# Autodesk Inventor assembly: sistema embebido
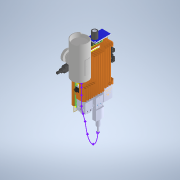
[picture p0: Inventor's stored thumbnail of the model, 180x180]
Saved by Autodesk Inventor 2021 (Build 250183000, 183)
## iProperties
Created: 2022-12-03
Part Number: sistema embebido
Document SubType Name: Assembly
Designer: user
Author: user
## Documents named in this file (9)
- D:\ESPOL\Tesis\3d proto\Total\sistema embebido.iam
- D:\ESPOL\Tesis\3d proto\Total\Assembly Raspberry Pi 4 B.iam
- D:\ESPOL\Tesis\3d proto\Total\Heat sink.ipt
- D:\ESPOL\Tesis\3d proto\Total\Heatsink Base.ipt
- D:\ESPOL\Tesis\3d proto\Total\MLX90640.ipt
- D:\ESPOL\Tesis\3d proto\Total\camara hd.ipt
- D:\ESPOL\Tesis\3d proto\Total\cable usb.ipt
- D:\ESPOL\Tesis\3d proto\Total\USB C.ipt
- D:\ESPOL\Tesis\3d proto\Total\jumper.ipt
## Components (21 placed, 8 different names)
1. Assembly Raspberry Pi 4 B:1 [sub-assembly] — Coincidencia:1, Coincidencia:2, Nivelación:1, Nivelación:2, Nivelación:3, Nivelación:4, Coincidencia:3, Coincidencia:4, Coincidencia:5, Coincidencia:10, Coincidencia:11, Coincidencia:17, Coincidencia:18, Coincidencia:19, Coincidencia:20, Coincidencia:21, Coincidencia:22, Coincidencia:23, Coincidencia:24, Coincidencia:25, Coincidencia:26, Coincidencia:27, Coincidencia:28, Coincidencia:29, Coincidencia:30, Coincidencia:31, Coincidencia:32, Coincidencia:33, Coincidencia:34, Coincidencia:35, Coincidencia:36
2. Heat sink:1 — Coincidencia:2, Nivelación:1, Nivelación:4
3. Heatsink Base:1 — Coincidencia:1, Nivelación:2, Nivelación:3, Coincidencia:37
4. MLX90640:1 — Coincidencia:3, Coincidencia:12, Coincidencia:13, Coincidencia:14, Coincidencia:15
5. camara hd:1 — Coincidencia:6, Coincidencia:37
6. cable usb:1 — Coincidencia:4, Coincidencia:5, Coincidencia:7
7. USB C:1 — Coincidencia:10, Coincidencia:11
8. jumper:1 — Coincidencia:15
9. jumper:2 — Coincidencia:14
10. jumper:3 — Coincidencia:13
11. jumper:4 — Coincidencia:23, Coincidencia:24
12. jumper:5 — Coincidencia:25, Coincidencia:26
13. jumper:6 — Coincidencia:27, Coincidencia:28
14. jumper:7 — Coincidencia:19, Coincidencia:20
15. jumper:8 — Coincidencia:12
16. jumper:9 — Coincidencia:21, Coincidencia:22
17. jumper:10 — Coincidencia:17, Coincidencia:18
18. jumper:11 — Coincidencia:31, Coincidencia:32
19. jumper:12 — Coincidencia:33, Coincidencia:34
20. jumper:13 — Coincidencia:35, Coincidencia:36
21. jumper:14 — Coincidencia:29, Coincidencia:30
## Relationships (40: Mate 36, Flush 4)
- Coincidencia:1 [Mate]: Assembly Raspberry Pi 4 B:1 ↔ Heatsink Base:1
- Coincidencia:2 [Mate]: Assembly Raspberry Pi 4 B:1 ↔ Heat sink:1
- Nivelación:1 [Flush]: Assembly Raspberry Pi 4 B:1 ↔ Heat sink:1
- Nivelación:2 [Flush]: Assembly Raspberry Pi 4 B:1 ↔ Heatsink Base:1
- Nivelación:3 [Flush]: Assembly Raspberry Pi 4 B:1 ↔ Heatsink Base:1
- Nivelación:4 [Flush]: Assembly Raspberry Pi 4 B:1 ↔ Heat sink:1
- Coincidencia:3 [Mate] (20 mm): Assembly Raspberry Pi 4 B:1 ↔ MLX90640:1
- Coincidencia:4 [Mate]: Assembly Raspberry Pi 4 B:1 ↔ cable usb:1
- Coincidencia:5 [Mate]: Assembly Raspberry Pi 4 B:1 ↔ cable usb:1
- Coincidencia:6 [Mate]: camara hd:1
- Coincidencia:7 [Mate]: cable usb:1
- Coincidencia:8 [Mate]
- Coincidencia:9 [Mate]
- Coincidencia:10 [Mate]: Assembly Raspberry Pi 4 B:1 ↔ USB C:1
- Coincidencia:11 [Mate]: Assembly Raspberry Pi 4 B:1 ↔ USB C:1
- Coincidencia:12 [Mate]: MLX90640:1 ↔ jumper:8
- Coincidencia:13 [Mate]: MLX90640:1 ↔ jumper:3
- Coincidencia:14 [Mate]: MLX90640:1 ↔ jumper:2
- Coincidencia:15 [Mate]: MLX90640:1 ↔ jumper:1
- Coincidencia:17 [Mate]: Assembly Raspberry Pi 4 B:1 ↔ jumper:10
- Coincidencia:18 [Mate]: Assembly Raspberry Pi 4 B:1 ↔ jumper:10
- Coincidencia:19 [Mate]: Assembly Raspberry Pi 4 B:1 ↔ jumper:7
- Coincidencia:20 [Mate]: Assembly Raspberry Pi 4 B:1 ↔ jumper:7
- Coincidencia:21 [Mate]: Assembly Raspberry Pi 4 B:1 ↔ jumper:9
- Coincidencia:22 [Mate]: Assembly Raspberry Pi 4 B:1 ↔ jumper:9
- Coincidencia:23 [Mate]: Assembly Raspberry Pi 4 B:1 ↔ jumper:4
- Coincidencia:24 [Mate]: Assembly Raspberry Pi 4 B:1 ↔ jumper:4
- Coincidencia:25 [Mate]: Assembly Raspberry Pi 4 B:1 ↔ jumper:5
- Coincidencia:26 [Mate]: Assembly Raspberry Pi 4 B:1 ↔ jumper:5
- Coincidencia:27 [Mate]: Assembly Raspberry Pi 4 B:1 ↔ jumper:6
- Coincidencia:28 [Mate]: Assembly Raspberry Pi 4 B:1 ↔ jumper:6
- Coincidencia:29 [Mate]: Assembly Raspberry Pi 4 B:1 ↔ jumper:14
- Coincidencia:30 [Mate]: Assembly Raspberry Pi 4 B:1 ↔ jumper:14
- Coincidencia:31 [Mate]: Assembly Raspberry Pi 4 B:1 ↔ jumper:11
- Coincidencia:32 [Mate]: Assembly Raspberry Pi 4 B:1 ↔ jumper:11
- Coincidencia:33 [Mate]: Assembly Raspberry Pi 4 B:1 ↔ jumper:12
- Coincidencia:34 [Mate]: Assembly Raspberry Pi 4 B:1 ↔ jumper:12
- Coincidencia:35 [Mate]: Assembly Raspberry Pi 4 B:1 ↔ jumper:13
- Coincidencia:36 [Mate]: Assembly Raspberry Pi 4 B:1 ↔ jumper:13
- Coincidencia:37 [Mate]: Heatsink Base:1 ↔ camara hd:1
